# Autodesk Inventor assembly: two part fix pilar assembly
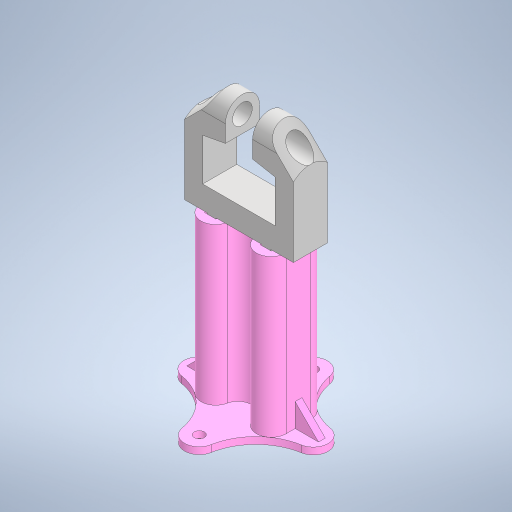
[picture p0: Inventor's stored thumbnail of the model, 512x512]
Saved by Autodesk Inventor 2024 (Build 280153000, 153)
## iProperties
Created: 2024-05-01
Part Number: two part fix pilar assembly
Document SubType Name: Assembly
Designer: compu
Author: compu
## Documents named in this file (3)
- C:\Users\compu\Documents\1Juan\1Facultad\9 Semestre\E1225 Taller de Sistemas Digitales\0Repository\BandTBS\Piezas\Partes 3D\Articulacion central\two part fix pilar assembly.iam
- C:\Users\compu\Documents\1Juan\1Facultad\9 Semestre\E1225 Taller de Sistemas Digitales\0Repository\BandTBS\Piezas\Partes 3D\Articulacion central\pilar soporte.ipt
- C:\Users\compu\Documents\1Juan\1Facultad\9 Semestre\E1225 Taller de Sistemas Digitales\0Repository\BandTBS\Piezas\Partes 3D\Articulacion central\pilar central pinza.ipt
## Components (2 placed, 2 different names)
1. pilar soporte:1 — Mate:1, Mate:3, Mate:4, Mate:7
2. pilar central pinza:1 — Mate:5, Flush:1, Mate:7
## Relationships (7: Mate 6, Flush 1)
- Mate:1: pilar soporte:1
- Mate:3: pilar soporte:1
- Mate:4: pilar soporte:1
- Mate:5: pilar central pinza:1
- Flush:1 (6 mm): pilar central pinza:1
- Mate:6
- Mate:7: pilar soporte:1 ↔ pilar central pinza:1
